# Autodesk Inventor assembly: Full Car Assembly
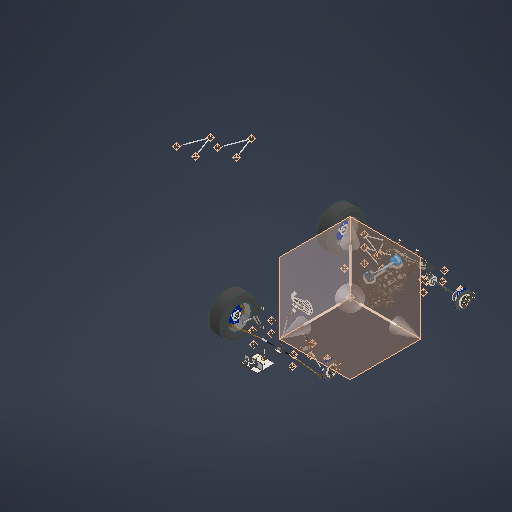
[picture p0: Inventor's stored thumbnail of the model, 512x512]
Saved by Autodesk Inventor 2026.1 (Build 301233000, 233)
## iProperties
Created: 2026-07-07
Part Number: Full Car Assembly
Document SubType Name: Assembly
Designer: share
Mass: 339781 g
Surface Area: 198029 cm^2
Volume: 256393 cm^3
Density: 1.32523 g/cm^3
Author: share
## Documents named in this file (36)
- C:\Users\share\OneDrive\Documents\Personal Projects\GOGO Kart\CAD\GOGO_KART_FSAE\Full Car Assembly.iam
- C:\Users\share\OneDrive\Documents\Personal Projects\GOGO Kart\CAD\GOGO_KART_FSAE\FrameV2\Frame\Frame 1780692296746.iam
- C:\Users\share\OneDrive\Documents\Personal Projects\GOGO Kart\CAD\GOGO_KART_FSAE\Drivetrain\honda-cbr600-f4i-engine-1.snapshot.3\Honda CBR600 F4i\Honda CBR600 F4i\Honda CBR600 F4i.ipt
- C:\Users\share\OneDrive\Documents\Personal Projects\GOGO Kart\CAD\GOGO_KART_FSAE\Shifter\crank.ipt
- C:\Users\share\OneDrive\Documents\Personal Projects\GOGO Kart\CAD\GOGO_KART_FSAE\Shifter\59935K71_Ball Joint Rod End\59935K71_Ball Joint Rod End\59935K71_Ball Joint Rod End.ipt
- C:\Users\share\OneDrive\Documents\Personal Projects\GOGO Kart\CAD\GOGO_KART_FSAE\Shifter\threadedtubeshort.ipt
- C:\Users\share\OneDrive\Documents\Personal Projects\GOGO Kart\CAD\GOGO_KART_FSAE\Shifter\ShifterBracket.ipt
- C:\Users\share\OneDrive\Documents\Personal Projects\GOGO Kart\CAD\GOGO_KART_FSAE\Shifter\BellCrank.ipt
- C:\Users\share\OneDrive\Documents\Personal Projects\GOGO Kart\CAD\GOGO_KART_FSAE\Shifter\Bearing.ipt
- C:\Users\share\OneDrive\Documents\Personal Projects\GOGO Kart\CAD\GOGO_KART_FSAE\Shifter\spacer.ipt
- C:\Users\share\OneDrive\Documents\Personal Projects\GOGO Kart\CAD\GOGO_KART_FSAE\Shifter\6045N121_Low-Carbon Steel Round Tube\6045N121_Low-Carbon Steel Round Tube\6045N121_Low-Carbon Steel Round Tube.ipt
- C:\Users\share\OneDrive\Documents\Inventor\Content Center Files\R2026\en-US\ISO 4032(2)\ISO 4032 - M5 - ISO.ipt
- C:\Users\share\OneDrive\Documents\Personal Projects\GOGO Kart\CAD\GOGO_KART_FSAE\Shifter\stickshift.ipt
- C:\Users\share\OneDrive\Documents\Personal Projects\GOGO Kart\CAD\GOGO_KART_FSAE\Shifter\stickplate.ipt
- C:\Users\share\OneDrive\Documents\Personal Projects\GOGO Kart\CAD\GOGO_KART_FSAE\Suspension\Hardware\ALLSTAR 0.5 in Rod End Bracket (Rough).ipt
- C:\Users\share\OneDrive\Documents\Personal Projects\GOGO Kart\CAD\GOGO_KART_FSAE\Drivetrain\Engine Mounting\Engine_Mount_Reference_Model_V1.ipt
- C:\Users\share\OneDrive\Documents\Personal Projects\GOGO Kart\CAD\GOGO_KART_FSAE\Drivetrain\Left_Engine_Mount_Assembly_V1.iam
- C:\Users\share\OneDrive\Documents\Personal Projects\GOGO Kart\CAD\GOGO_KART_FSAE\Drivetrain\Right_Lower_Engine_Mount_Assembly_V1.iam
- C:\Users\share\OneDrive\Documents\Personal Projects\GOGO Kart\CAD\GOGO_KART_FSAE\Suspension\SpringSetup\largebracket.ipt
- C:\Users\share\OneDrive\Documents\Personal Projects\GOGO Kart\CAD\GOGO_KART_FSAE\Suspension\SpringSetup\ShockAbsorber.ipt
- C:\Users\share\OneDrive\Documents\Personal Projects\GOGO Kart\CAD\GOGO_KART_FSAE\Suspension\SpringSetup\RockerFront.ipt
- C:\Users\share\OneDrive\Documents\Personal Projects\GOGO Kart\CAD\GOGO_KART_FSAE\Suspension\SpringSetup\sus_rods.ipt
- C:\Users\share\OneDrive\Documents\Personal Projects\GOGO Kart\CAD\GOGO_KART_FSAE\Suspension\Suspension Arms\Suspension Rod Ends\5-8 Rod End Assembly.iam
- C:\Users\share\OneDrive\Documents\Personal Projects\GOGO Kart\CAD\GOGO_KART_FSAE\Suspension\SpringSetup\RockerRear.ipt
- C:\Users\share\OneDrive\Documents\Personal Projects\GOGO Kart\CAD\GOGO_KART_FSAE\Suspension\SpringSetup\susrod_rear.ipt
- C:\Users\share\OneDrive\Documents\Personal Projects\GOGO Kart\CAD\GOGO_KART_FSAE\Steering\SteeringAssy.iam
- C:\Users\share\OneDrive\Documents\Personal Projects\GOGO Kart\CAD\GOGO_KART_FSAE\Steering\steeringmountplate.ipt
- C:\Users\share\OneDrive\Documents\Personal Projects\GOGO Kart\CAD\GOGO_KART_FSAE\Steering\steeringbracket.ipt
- C:\Users\share\OneDrive\Documents\Personal Projects\GOGO Kart\CAD\GOGO_KART_FSAE\Steering\rackbracket.ipt
- C:\Users\share\OneDrive\Documents\Personal Projects\GOGO Kart\CAD\GOGO_KART_FSAE\Steering\rackmountplate.ipt
- C:\Users\share\OneDrive\Documents\Personal Projects\GOGO Kart\CAD\GOGO_KART_FSAE\Drivetrain\Diff_Assembly_V1.iam
- C:\Users\share\OneDrive\Documents\Personal Projects\GOGO Kart\CAD\GOGO_KART_FSAE\Drivetrain\CV Axles\Porsche_912_Standard_CV_Axle_Assembly.iam
- C:\Users\share\OneDrive\Documents\Personal Projects\GOGO Kart\CAD\GOGO_KART_FSAE\Suspension\REAL Upright\V2\Upright_Assembly_V2.iam
- C:\Users\share\Downloads\Driver CAD Model.iam
- C:\Users\share\OneDrive\Documents\Personal Projects\GOGO Kart\CAD\GOGO_KART_FSAE\Pedal Box\Pedal_Box_V2_Test\Pedalbox_V2_Assembly.iam
- C:\Users\share\OneDrive\Documents\Personal Projects\GOGO Kart\CAD\GOGO_KART_FSAE\Suspension\Suspension_Arm_V2\Suspenion_Arm_Assembly_V2.iam
## Components (93 placed, 35 different names)
1. Porsche_912_Standard_CV_Axle_Assembly:1 [sub-assembly] — Mate:66, Rigid:6, Mate:71
2. Porsche_912_Standard_CV_Axle_Assembly:2 [sub-assembly] — Mate:67, Mate:68, Mate:70
3. Upright_Assembly_V2:1 [sub-assembly] — Angle:33
4. Upright_Assembly_V2:2 [sub-assembly] — Angle:32
5. Upright_Assembly_V2:3 [sub-assembly] — Angle:35, Mate:70
6. Upright_Assembly_V2:4 [sub-assembly] — Angle:34, Mate:71
7. Driver CAD Model:1 [sub-assembly]
8. Pedalbox_V2_Assembly:1 [sub-assembly] — Tangent:36, Tangent:37, Mate:72
9. Suspenion_Arm_Assembly_V2:1 [sub-assembly] — Mate:73, Mate:74
10. Suspenion_Arm_Assembly_V2:2 [sub-assembly] — Mate:75, Mate:76
11. Suspenion_Arm_Assembly_V2:3 [sub-assembly]
12. Suspenion_Arm_Assembly_V2:4 [sub-assembly]
13. Porsche_912_Standard_CV_Axle_Assembly:3 [sub-assembly]
14. Frame 1780692296746:1 [sub-assembly] — Flush:1, Flush:2, Flush:3, Tangent:1, Tangent:2, Front Left: LF Floor Mate, Front Left: LF Front Mate, Front Left: LF Tangent Mate, Front Left: LR Floor Mate, Front Left: LR Front Mate, Front Left: LR Tangent Mate, Front Left: UF Floor Mate, Front Left: UF Front Mate, Front Left: UF Tangent Mate, Front Left: UR Floor Mate, Front Left: UR Front Mate, Front Left: UR Tangent Mate, Rear Left: LF Floor Mate, Rear Left: LF Front Mate, Rear Left: LF Tangent Mate, Rear Left: LR Floor Mate, Rear Left: LR Front Mate, Rear Left: LR Tangent Mate, Rear Left: UF Floor Mate, Rear Left: UF Front Mate, Rear Left: UF Tangent Mate, Rear Left: UR Floor Mate, Rear Left: UR Front Mate, Rear Left: UR Tangent Mate, Front Right: LF Floor Mate, Front Right: LF Front Mate, Front Right: LF Tangent  Mate, Front Right: LR Floor Mate, Front Right: LR Front Mate, Front Right: LR Tangent  Mate, Front Right: UF Floor Mate, Front Right: UF Front Mate, Front Right: UF Tangent Mate, Front Right: UR Floor Mate, Front Right: UR Front Mate, Front Right: UR Tangent  Mate, Rear Right: LF Floor Mate, Rear Right: LF Front Mate, Rear Right: LF Tangent Mate, Rear Right: LR Floor Mate, Rear Right: LR Front Mate, Rear Right: LR Tangent Mate, Rear Right: UR Floor Mate, Rear Right: UR Front Mate, Rear Ritgh: UR Tangent Mate, Rear Right: UF Floor Mate, Rear Right: UF Front Mate, Rear Rigth: UF Tangent Mate, Engine Reference Horizontal Mate, Engine Reference Vertical Mate, Insert:3, Angle:2, Insert:4, Angle:4, Angle:6, Angle:7, Insert:6, Insert:7, Tangent:19, Mate:39, Tangent:20, Mate:40, Tangent:21, Tangent:22, Tangent:23, Tangent:24, Tangent:25, Tangent:28, Tangent:30, Tangent:31, Mate:54, Tangent:33, Tangent:34, Mate:69, Tangent:35, Tangent:36, Tangent:37
15. stickshift:1 — Rigid:4
16. stickplate:1 — Rigid:4, Tangent:2
17. crank:1 — Insert:2
18. 59935K71_Ball Joint Rod End:1 — Rotational:2, Angle:1, Rotational:6
19. 59935K71_Ball Joint Rod End:3 — Insert:2, Rotational:1, Angle:1
20. threadedtubeshort:1 — Rotational:1, Rotational:2
21. ShifterBracket:1 — Rigid:1, Tangent:1
22. BellCrank:1 — Rotational:3, Rotational:6
23. Bearing:1 — Rotational:3, Rotational:4, Rotational:5
24. spacer:1 — Rigid:1, Rotational:4
25. spacer:2 — Rotational:5
26. 6045N121_Low-Carbon Steel Round Tube:1 — Rigid:2, Rigid:3
27. ISO 4032 M5:1 — Rigid:3
28. ISO 4032 M5:2 — Rigid:2
29. 5-8 Rod End Assembly:7 [sub-assembly] — Rotational:77, Angle:25
30. 5-8 Rod End Assembly:8 [sub-assembly] — Rotational:78, Angle:27
31. ALLSTAR 0.5 in Rod End Bracket (Rough):23 — Rotational:78, Angle:27
32. 5-8 Rod End Assembly:3 [sub-assembly] — Rotational:57, Rotational:59
33. 5-8 Rod End Assembly:4 [sub-assembly] — Rotational:58, Rotational:61, Angle:15, Angle:16
34. ALLSTAR 0.5 in Rod End Bracket (Rough):20 — Angle:12
35. ALLSTAR 0.5 in Rod End Bracket (Rough):21 — Rotational:61, Angle:15
36. 5-8 Rod End Assembly:5 [sub-assembly] — Rotational:69, Angle:20
37. 5-8 Rod End Assembly:6 [sub-assembly] — Angle:19, Rotational:70
38. ALLSTAR 0.5 in Rod End Bracket (Rough):22 — Rotational:69, Angle:20, Angle:21
39. largebracket:8 — Tangent:30, Angle:22, Mate:50, Mate:51, Rotational:71
40. largebracket:9 — Angle:23, Tangent:31, Mate:52, Rotational:72, Rotational:73
41. RockerRear:3 — Rotational:72, Angle:24, Rotational:74, Rotational:77, Angle:25
42. RockerRear:4 — Rotational:73, Angle:24
43. susrod_rear:2
44. largebracket:7 — Mate:49, Angle:17, Tangent:28, Rotational:62
45. ShockAbsorber:3 — Rotational:62, Rotational:65
46. ShockAbsorber:4 — Rotational:71, Rotational:74
47. RockerFront:4 — Rotational:64, Angle:18, Rotational:65, Angle:21, Rotational:70
48. RockerFront:5 — Rotational:63, Angle:18, Angle:19
49. sus_rods:2
50. largebracket:5 — Tangent:24, Angle:9, Mate:46, Mate:47, Rotational:55, Angle:22
51. largebracket:6 — Angle:10, Tangent:25, Mate:48, Rotational:53, Rotational:54, Angle:23
52. RockerRear:1 — Rotational:53, Angle:11, Rotational:59, Angle:16
53. RockerRear:2 — Rotational:54, Angle:11, Rotational:56
54. ShockAbsorber:2 — Rotational:55, Rotational:56
55. susrod_rear:1 — Rotational:57, Rotational:58
56. largebracket:1 — Tangent:21, Mate:41, Mate:42, Rotational:42, Rotational:43
57. largebracket:2 — Tangent:22, Mate:43, Mate:44, Angle:17, Rotational:63, Rotational:64
58. largebracket:4 — Tangent:23, Mate:45, Rotational:41
59. ShockAbsorber:1 — Rotational:41, Rotational:44
60. RockerFront:2 — Rotational:42, Angle:8, Rotational:44, Angle:12
61. RockerFront:3 — Rotational:43, Angle:8
62. sus_rods:1
63. ALLSTAR 0.5 in Rod End Bracket (Rough):1 — Front Left: LF Floor Mate, Front Left: LF Front Mate, Front Left: LF Tangent Mate
64. ALLSTAR 0.5 in Rod End Bracket (Rough):2 — Front Left: LR Floor Mate, Front Left: LR Front Mate, Front Left: LR Tangent Mate
65. ALLSTAR 0.5 in Rod End Bracket (Rough):3 — Front Left: UF Floor Mate, Front Left: UF Front Mate, Front Left: UF Tangent Mate, Mate:42
66. ALLSTAR 0.5 in Rod End Bracket (Rough):4 — Front Left: UR Floor Mate, Front Left: UR Front Mate, Front Left: UR Tangent Mate
67. ALLSTAR 0.5 in Rod End Bracket (Rough):5 — Rear Left: LF Floor Mate, Rear Left: LF Front Mate, Rear Left: LF Tangent Mate
68. ALLSTAR 0.5 in Rod End Bracket (Rough):6 — Rear Left: UF Floor Mate, Rear Left: UF Front Mate, Rear Left: UF Tangent Mate
69. ALLSTAR 0.5 in Rod End Bracket (Rough):7 — Rear Left: UR Floor Mate, Rear Left: UR Front Mate, Rear Left: UR Tangent Mate, Angle:9, Angle:10
70. ALLSTAR 0.5 in Rod End Bracket (Rough):8 — Rear Left: LR Floor Mate, Rear Left: LR Front Mate, Rear Left: LR Tangent Mate
71. ALLSTAR 0.5 in Rod End Bracket (Rough):9 — Front Right: LF Floor Mate, Front Right: LF Front Mate, Front Right: LF Tangent  Mate
72. ALLSTAR 0.5 in Rod End Bracket (Rough):10 — Front Right: LR Floor Mate, Front Right: LR Front Mate, Front Right: LR Tangent  Mate
73. ALLSTAR 0.5 in Rod End Bracket (Rough):11 — Front Right: UR Floor Mate, Front Right: UR Front Mate, Front Right: UR Tangent  Mate
74. ALLSTAR 0.5 in Rod End Bracket (Rough):12 — Front Right: UF Floor Mate, Front Right: UF Front Mate, Front Right: UF Tangent Mate, Mate:44
75. ALLSTAR 0.5 in Rod End Bracket (Rough):13 — Rear Right: LF Floor Mate, Rear Right: LF Front Mate, Rear Right: LF Tangent Mate, Mate:76
76. ALLSTAR 0.5 in Rod End Bracket (Rough):14 — Rear Right: LR Floor Mate, Rear Right: LR Front Mate, Rear Right: LR Tangent Mate, Mate:75
77. ALLSTAR 0.5 in Rod End Bracket (Rough):15 — Rear Right: UR Floor Mate, Rear Right: UR Front Mate, Rear Ritgh: UR Tangent Mate, Mate:73
78. ALLSTAR 0.5 in Rod End Bracket (Rough):16 — Rear Right: UF Floor Mate, Rear Right: UF Front Mate, Rear Rigth: UF Tangent Mate, Mate:74
79. Honda CBR600 F4i:1 — Insert:5, Angle:4
80. Engine_Mount_Reference_Model_V1:1 — Engine Reference Horizontal Mate, Engine Reference Vertical Mate
81. ALLSTAR 0.5 in Rod End Bracket (Rough):18 — Tangent:19, Mate:39
82. ALLSTAR 0.5 in Rod End Bracket (Rough):19 — Tangent:20, Mate:40
83. Left_Engine_Mount_Assembly_V1:1 [sub-assembly] — Insert:3, Angle:2, Angle:3, Insert:5
84. Left_Engine_Mount_Assembly_V1:2 [sub-assembly] — Insert:4, Angle:3
85. Right_Lower_Engine_Mount_Assembly_V1:1 [sub-assembly] — Angle:6, Insert:7
86. Right_Lower_Engine_Mount_Assembly_V1:2 [sub-assembly] — Angle:7, Insert:6
87. Diff_Assembly_V1:1 [sub-assembly] — Angle:31, Mate:66, Rigid:6, Mate:67, Mate:68, Mate:69, Tangent:35
88. SteeringAssy:1 [sub-assembly] — Rotational:83, Angle:28, Mate:63, Angle:29, Angle:30
89. steeringmountplate:1 — Mate:53, Mate:54, Mate:55, Rotational:79, Rotational:80
90. steeringbracket:1 — Rotational:79, Rotational:80, Rotational:83
91. rackmountplate:1 — Tangent:33, Tangent:34, Mate:56, Rotational:84, Mate:62, Angle:28, Rotational:85, Mate:64, Angle:29, Angle:30
92. rackbracket:2 — Rotational:84, Mate:62, Mate:63
93. rackbracket:3 — Rotational:85, Mate:64
## Relationships (183: Mate 57, RevoluteJoint 39, Tangent 33, Angle 31, Flush 12, Insert 6, WeldJoint 5)
- Flush:1: Frame 1780692296746:1
- Flush:2: Frame 1780692296746:1
- Flush:3: Frame 1780692296746:1
- Insert:2: crank:1 ↔ 59935K71_Ball Joint Rod End:3
- Rotational:1 [RevoluteJoint]: 59935K71_Ball Joint Rod End:3 ↔ threadedtubeshort:1
- Rotational:2 [RevoluteJoint]: 59935K71_Ball Joint Rod End:1 ↔ threadedtubeshort:1
- Angle:1 (90 deg): 59935K71_Ball Joint Rod End:1 ↔ 59935K71_Ball Joint Rod End:3
- Rigid:1 [WeldJoint]: ShifterBracket:1 ↔ spacer:1
- Rotational:3 [RevoluteJoint]: BellCrank:1 ↔ Bearing:1
- Rotational:4 [RevoluteJoint]: Bearing:1 ↔ spacer:1
- Rotational:5 [RevoluteJoint]: Bearing:1 ↔ spacer:2
- Rotational:6 [RevoluteJoint]: 59935K71_Ball Joint Rod End:1 ↔ BellCrank:1
- Tangent:1: Frame 1780692296746:1 ↔ ShifterBracket:1
- Rigid:2 [WeldJoint]: 6045N121_Low-Carbon Steel Round Tube:1 ↔ ISO 4032 M5:2
- Rigid:3 [WeldJoint]: 6045N121_Low-Carbon Steel Round Tube:1 ↔ ISO 4032 M5:1
- Rigid:4 [WeldJoint]: stickshift:1 ↔ stickplate:1
- Tangent:2: Frame 1780692296746:1 ↔ stickplate:1
- Front Left: LF Floor Mate [Mate] (200 mm): Frame 1780692296746:1 ↔ ALLSTAR 0.5 in Rod End Bracket (Rough):1
- Front Left: LF Front Mate [Flush] (350 mm): Frame 1780692296746:1 ↔ ALLSTAR 0.5 in Rod End Bracket (Rough):1
- Front Left: LF Tangent Mate [Tangent]: Frame 1780692296746:1 ↔ ALLSTAR 0.5 in Rod End Bracket (Rough):1
- Front Left: LR Floor Mate [Mate] (200 mm): Frame 1780692296746:1 ↔ ALLSTAR 0.5 in Rod End Bracket (Rough):2
- Front Left: LR Front Mate [Flush] (610 mm): Frame 1780692296746:1 ↔ ALLSTAR 0.5 in Rod End Bracket (Rough):2
- Front Left: LR Tangent Mate [Tangent]: Frame 1780692296746:1 ↔ ALLSTAR 0.5 in Rod End Bracket (Rough):2
- Front Left: UF Floor Mate [Mate] (350 mm): Frame 1780692296746:1 ↔ ALLSTAR 0.5 in Rod End Bracket (Rough):3
- Front Left: UF Front Mate [Flush] (360 mm): Frame 1780692296746:1 ↔ ALLSTAR 0.5 in Rod End Bracket (Rough):3
- Front Left: UF Tangent Mate [Tangent]: Frame 1780692296746:1 ↔ ALLSTAR 0.5 in Rod End Bracket (Rough):3
- Front Left: UR Floor Mate [Mate] (350 mm): Frame 1780692296746:1 ↔ ALLSTAR 0.5 in Rod End Bracket (Rough):4
- Front Left: UR Front Mate [Flush] (620 mm): Frame 1780692296746:1 ↔ ALLSTAR 0.5 in Rod End Bracket (Rough):4
- Front Left: UR Tangent Mate [Tangent]: Frame 1780692296746:1 ↔ ALLSTAR 0.5 in Rod End Bracket (Rough):4
- Rear Left: LF Floor Mate [Mate] (200 mm): Frame 1780692296746:1 ↔ ALLSTAR 0.5 in Rod End Bracket (Rough):5
- Rear Left: LF Front Mate [Flush] (2180 mm): Frame 1780692296746:1 ↔ ALLSTAR 0.5 in Rod End Bracket (Rough):5
- Rear Left: LF Tangent Mate [Tangent]: Frame 1780692296746:1 ↔ ALLSTAR 0.5 in Rod End Bracket (Rough):5
- Rear Left: LR Floor Mate [Mate] (200 mm): Frame 1780692296746:1 ↔ ALLSTAR 0.5 in Rod End Bracket (Rough):8
- Rear Left: LR Front Mate [Flush] (2440 mm): Frame 1780692296746:1 ↔ ALLSTAR 0.5 in Rod End Bracket (Rough):8
- Rear Left: LR Tangent Mate [Tangent]: Frame 1780692296746:1 ↔ ALLSTAR 0.5 in Rod End Bracket (Rough):8
- Rear Left: UF Floor Mate [Mate] (350 mm): Frame 1780692296746:1 ↔ ALLSTAR 0.5 in Rod End Bracket (Rough):6
- Rear Left: UF Front Mate [Flush] (2180 mm): Frame 1780692296746:1 ↔ ALLSTAR 0.5 in Rod End Bracket (Rough):6
- Rear Left: UF Tangent Mate [Tangent]: Frame 1780692296746:1 ↔ ALLSTAR 0.5 in Rod End Bracket (Rough):6
- Rear Left: UR Floor Mate [Mate] (350 mm): Frame 1780692296746:1 ↔ ALLSTAR 0.5 in Rod End Bracket (Rough):7
- Rear Left: UR Front Mate [Flush] (2440 mm): Frame 1780692296746:1 ↔ ALLSTAR 0.5 in Rod End Bracket (Rough):7
- Rear Left: UR Tangent Mate [Tangent]: Frame 1780692296746:1 ↔ ALLSTAR 0.5 in Rod End Bracket (Rough):7
- Front Right: LF Floor Mate [Mate] (200 mm): Frame 1780692296746:1 ↔ ALLSTAR 0.5 in Rod End Bracket (Rough):9
- Front Right: LF Front Mate [Mate] (-350 mm): Frame 1780692296746:1 ↔ ALLSTAR 0.5 in Rod End Bracket (Rough):9
- Front Right: LF Tangent  Mate [Tangent]: Frame 1780692296746:1 ↔ ALLSTAR 0.5 in Rod End Bracket (Rough):9
- Front Right: LR Floor Mate [Mate] (200 mm): Frame 1780692296746:1 ↔ ALLSTAR 0.5 in Rod End Bracket (Rough):10
- Front Right: LR Front Mate [Mate] (-610 mm): Frame 1780692296746:1 ↔ ALLSTAR 0.5 in Rod End Bracket (Rough):10
- Front Right: LR Tangent  Mate [Tangent]: Frame 1780692296746:1 ↔ ALLSTAR 0.5 in Rod End Bracket (Rough):10
- Front Right: UF Floor Mate [Mate] (350 mm): Frame 1780692296746:1 ↔ ALLSTAR 0.5 in Rod End Bracket (Rough):12
- Front Right: UF Front Mate [Mate] (-360 mm): Frame 1780692296746:1 ↔ ALLSTAR 0.5 in Rod End Bracket (Rough):12
- Front Right: UF Tangent Mate [Tangent]: Frame 1780692296746:1 ↔ ALLSTAR 0.5 in Rod End Bracket (Rough):12
- Front Right: UR Floor Mate [Mate] (350 mm): Frame 1780692296746:1 ↔ ALLSTAR 0.5 in Rod End Bracket (Rough):11
- Front Right: UR Front Mate [Mate] (-620 mm): Frame 1780692296746:1 ↔ ALLSTAR 0.5 in Rod End Bracket (Rough):11
- Front Right: UR Tangent  Mate [Tangent]: Frame 1780692296746:1 ↔ ALLSTAR 0.5 in Rod End Bracket (Rough):11
- Rear Right: LF Floor Mate [Mate] (200 mm): Frame 1780692296746:1 ↔ ALLSTAR 0.5 in Rod End Bracket (Rough):13
- Rear Right: LF Front Mate [Mate] (-2180 mm): Frame 1780692296746:1 ↔ ALLSTAR 0.5 in Rod End Bracket (Rough):13
- Rear Right: LF Tangent Mate [Tangent]: Frame 1780692296746:1 ↔ ALLSTAR 0.5 in Rod End Bracket (Rough):13
- Rear Right: LR Floor Mate [Mate] (200 mm): Frame 1780692296746:1 ↔ ALLSTAR 0.5 in Rod End Bracket (Rough):14
- Rear Right: LR Front Mate [Mate] (-2440 mm): Frame 1780692296746:1 ↔ ALLSTAR 0.5 in Rod End Bracket (Rough):14
- Rear Right: LR Tangent Mate [Tangent]: Frame 1780692296746:1 ↔ ALLSTAR 0.5 in Rod End Bracket (Rough):14
- Rear Right: UR Floor Mate [Mate] (350 mm): Frame 1780692296746:1 ↔ ALLSTAR 0.5 in Rod End Bracket (Rough):15
- Rear Right: UR Front Mate [Mate] (-2440 mm): Frame 1780692296746:1 ↔ ALLSTAR 0.5 in Rod End Bracket (Rough):15
- Rear Ritgh: UR Tangent Mate [Tangent]: Frame 1780692296746:1 ↔ ALLSTAR 0.5 in Rod End Bracket (Rough):15
- Rear Right: UF Floor Mate [Mate] (350 mm): Frame 1780692296746:1 ↔ ALLSTAR 0.5 in Rod End Bracket (Rough):16
- Rear Right: UF Front Mate [Mate] (-2180 mm): Frame 1780692296746:1 ↔ ALLSTAR 0.5 in Rod End Bracket (Rough):16
- Rear Rigth: UF Tangent Mate [Tangent]: Frame 1780692296746:1 ↔ ALLSTAR 0.5 in Rod End Bracket (Rough):16
- Engine Reference Horizontal Mate [Mate] (30 mm): Frame 1780692296746:1 ↔ Engine_Mount_Reference_Model_V1:1
- Engine Reference Vertical Mate [Flush] (400 mm): Frame 1780692296746:1 ↔ Engine_Mount_Reference_Model_V1:1
- Insert:3: Frame 1780692296746:1 ↔ Left_Engine_Mount_Assembly_V1:1
- Angle:2 (0 deg): Frame 1780692296746:1 ↔ Left_Engine_Mount_Assembly_V1:1
- Insert:4: Frame 1780692296746:1 ↔ Left_Engine_Mount_Assembly_V1:2
- Angle:3 (0 deg): Left_Engine_Mount_Assembly_V1:1 ↔ Left_Engine_Mount_Assembly_V1:2
- Insert:5: Honda CBR600 F4i:1 ↔ Left_Engine_Mount_Assembly_V1:1
- Angle:4 (0 deg): Frame 1780692296746:1 ↔ Honda CBR600 F4i:1
- Angle:6 (0 deg): Frame 1780692296746:1 ↔ Right_Lower_Engine_Mount_Assembly_V1:1
- Angle:7 (0 deg): Frame 1780692296746:1 ↔ Right_Lower_Engine_Mount_Assembly_V1:2
- Insert:6: Frame 1780692296746:1 ↔ Right_Lower_Engine_Mount_Assembly_V1:2
- Insert:7: Frame 1780692296746:1 ↔ Right_Lower_Engine_Mount_Assembly_V1:1
- Tangent:19: Frame 1780692296746:1 ↔ ALLSTAR 0.5 in Rod End Bracket (Rough):18
- Mate:39 (400 mm): Frame 1780692296746:1 ↔ ALLSTAR 0.5 in Rod End Bracket (Rough):18
- Tangent:20: Frame 1780692296746:1 ↔ ALLSTAR 0.5 in Rod End Bracket (Rough):19
- Mate:40 (450 mm): Frame 1780692296746:1 ↔ ALLSTAR 0.5 in Rod End Bracket (Rough):19
- Tangent:21: Frame 1780692296746:1 ↔ largebracket:1
- Mate:41 (350 mm): largebracket:1
- Mate:42 (-105 mm): largebracket:1 ↔ ALLSTAR 0.5 in Rod End Bracket (Rough):3
- Tangent:22: Frame 1780692296746:1 ↔ largebracket:2
- Mate:43 (350 mm): largebracket:2
- Mate:44 (145 mm): largebracket:2 ↔ ALLSTAR 0.5 in Rod End Bracket (Rough):12
- Tangent:23: Frame 1780692296746:1 ↔ largebracket:4
- Mate:45 (590 mm): largebracket:4
- Rotational:41 [RevoluteJoint] (-9 mm): largebracket:4 ↔ ShockAbsorber:1
- Rotational:42 [RevoluteJoint]: largebracket:1 ↔ RockerFront:2
- Rotational:43 [RevoluteJoint]: largebracket:1 ↔ RockerFront:3
- Angle:8 (0 deg): RockerFront:2 ↔ RockerFront:3
- Rotational:44 [RevoluteJoint] (6.5 mm): ShockAbsorber:1 ↔ RockerFront:2
- Tangent:24: Frame 1780692296746:1 ↔ largebracket:5
- Angle:9 (0 deg): largebracket:5 ↔ ALLSTAR 0.5 in Rod End Bracket (Rough):7
- Mate:46 (-846 mm): largebracket:5
- Mate:47 (120 mm): largebracket:5
- Angle:10 (180 deg): largebracket:6 ↔ ALLSTAR 0.5 in Rod End Bracket (Rough):7
- Tangent:25: Frame 1780692296746:1 ↔ largebracket:6
- Mate:48 (280 mm): largebracket:6
- Rotational:53 [RevoluteJoint]: largebracket:6 ↔ RockerRear:1
- Rotational:54 [RevoluteJoint]: largebracket:6 ↔ RockerRear:2
- Angle:11 (0 deg): RockerRear:1 ↔ RockerRear:2
- Rotational:55 [RevoluteJoint] (-8.5 mm): largebracket:5 ↔ ShockAbsorber:2
- Rotational:56 [RevoluteJoint] (6 mm): RockerRear:2 ↔ ShockAbsorber:2
- Rotational:57 [RevoluteJoint] (2 mm): 5-8 Rod End Assembly:3 ↔ susrod_rear:1
- Rotational:58 [RevoluteJoint] (-2 mm): 5-8 Rod End Assembly:4 ↔ susrod_rear:1
- Rotational:59 [RevoluteJoint] (6.5 mm): 5-8 Rod End Assembly:3 ↔ RockerRear:1
- Angle:12 (0 deg): ALLSTAR 0.5 in Rod End Bracket (Rough):20 ↔ RockerFront:2
- Rotational:61 [RevoluteJoint]: 5-8 Rod End Assembly:4 ↔ ALLSTAR 0.5 in Rod End Bracket (Rough):21
- Angle:15 (0 deg): 5-8 Rod End Assembly:4 ↔ ALLSTAR 0.5 in Rod End Bracket (Rough):21
- Angle:16 (0 deg): 5-8 Rod End Assembly:4 ↔ RockerRear:1
- Mate:49 (590 mm): largebracket:7
- Angle:17 (180 deg): largebracket:7 ↔ largebracket:2
- Tangent:28: Frame 1780692296746:1 ↔ largebracket:7
- Rotational:62 [RevoluteJoint] (-9 mm): largebracket:7 ↔ ShockAbsorber:3
- Rotational:63 [RevoluteJoint]: RockerFront:5 ↔ largebracket:2
- Rotational:64 [RevoluteJoint]: RockerFront:4 ↔ largebracket:2
- Angle:18 (0 deg): RockerFront:4 ↔ RockerFront:5
- Rotational:65 [RevoluteJoint] (6.5 mm): ShockAbsorber:3 ↔ RockerFront:4
- [RevoluteJoint] (-2 mm): 5-8 Rod End Assembly:5 ↔ sus_rods:2
- [RevoluteJoint] (2 mm): 5-8 Rod End Assembly:6 ↔ sus_rods:2
- Angle:19 (0 deg): 5-8 Rod End Assembly:6 ↔ RockerFront:5
- Rotational:69 [RevoluteJoint]: 5-8 Rod End Assembly:5 ↔ ALLSTAR 0.5 in Rod End Bracket (Rough):22
- Angle:20 (0 deg): 5-8 Rod End Assembly:5 ↔ ALLSTAR 0.5 in Rod End Bracket (Rough):22
- Angle:21 (0 deg): ALLSTAR 0.5 in Rod End Bracket (Rough):22 ↔ RockerFront:4
- Rotational:70 [RevoluteJoint] (6.5 mm): 5-8 Rod End Assembly:6 ↔ RockerFront:4
- Tangent:30: Frame 1780692296746:1 ↔ largebracket:8
- Angle:22 (0 deg): largebracket:8 ↔ largebracket:5
- Mate:50 (-846 mm): largebracket:8
- Mate:51 (-120 mm): largebracket:8
- Angle:23 (0 deg): largebracket:9 ↔ largebracket:6
- Tangent:31: Frame 1780692296746:1 ↔ largebracket:9
- Mate:52 (-280 mm): largebracket:9
- Rotational:71 [RevoluteJoint] (-8.5 mm): largebracket:8 ↔ ShockAbsorber:4
- Rotational:72 [RevoluteJoint]: largebracket:9 ↔ RockerRear:3
- Rotational:73 [RevoluteJoint]: largebracket:9 ↔ RockerRear:4
- Angle:24 (0 deg): RockerRear:3 ↔ RockerRear:4
- Rotational:74 [RevoluteJoint] (6.5 mm): RockerRear:3 ↔ ShockAbsorber:4
- [RevoluteJoint] (2 mm): 5-8 Rod End Assembly:7 ↔ susrod_rear:2
- [RevoluteJoint] (-2 mm): 5-8 Rod End Assembly:8 ↔ susrod_rear:2
- Rotational:77 [RevoluteJoint] (6 mm): 5-8 Rod End Assembly:7 ↔ RockerRear:3
- Angle:25 (0 deg): 5-8 Rod End Assembly:7 ↔ RockerRear:3
- Rotational:78 [RevoluteJoint]: 5-8 Rod End Assembly:8 ↔ ALLSTAR 0.5 in Rod End Bracket (Rough):23
- Angle:27 (0 deg): 5-8 Rod End Assembly:8 ↔ ALLSTAR 0.5 in Rod End Bracket (Rough):23
- Mate:53 (-60 mm): steeringmountplate:1
- Mate:54: Frame 1780692296746:1 ↔ steeringmountplate:1
- Mate:55 (697 mm): steeringmountplate:1
- Rotational:79 [RevoluteJoint]: steeringmountplate:1 ↔ steeringbracket:1
- Rotational:80 [RevoluteJoint]: steeringmountplate:1 ↔ steeringbracket:1
- Tangent:33: Frame 1780692296746:1 ↔ rackmountplate:1
- Tangent:34: Frame 1780692296746:1 ↔ rackmountplate:1
- Mate:56 (-70 mm): rackmountplate:1
- Rotational:83 [RevoluteJoint]: SteeringAssy:1 ↔ steeringbracket:1
- Rotational:84 [RevoluteJoint]: rackmountplate:1 ↔ rackbracket:2
- Mate:62: rackmountplate:1 ↔ rackbracket:2
- Angle:28 (180 deg): SteeringAssy:1 ↔ rackmountplate:1
- Mate:63: SteeringAssy:1 ↔ rackbracket:2
- Rotational:85 [RevoluteJoint]: rackmountplate:1 ↔ rackbracket:3
- Mate:64: rackmountplate:1 ↔ rackbracket:3
- Angle:29 (173 deg): SteeringAssy:1 ↔ rackmountplate:1
- Angle:30 (187 deg): SteeringAssy:1 ↔ rackmountplate:1
- Angle:31 (0 deg): Diff_Assembly_V1:1
- Mate:66: Porsche_912_Standard_CV_Axle_Assembly:1 ↔ Diff_Assembly_V1:1
- Rigid:6 [WeldJoint]: Porsche_912_Standard_CV_Axle_Assembly:1 ↔ Diff_Assembly_V1:1
- Mate:67: Porsche_912_Standard_CV_Axle_Assembly:2 ↔ Diff_Assembly_V1:1
- Mate:68 (250 mm): Porsche_912_Standard_CV_Axle_Assembly:2 ↔ Diff_Assembly_V1:1
- Mate:69: Frame 1780692296746:1 ↔ Diff_Assembly_V1:1
- Tangent:35: Frame 1780692296746:1 ↔ Diff_Assembly_V1:1
- Angle:32 (180 deg): Upright_Assembly_V2:2
- Angle:33 (0 deg): Upright_Assembly_V2:1
- Angle:34 (0 deg): Upright_Assembly_V2:4
- Angle:35 (180 deg): Upright_Assembly_V2:3
- Mate:70: Porsche_912_Standard_CV_Axle_Assembly:2 ↔ Upright_Assembly_V2:3
- Mate:71: Porsche_912_Standard_CV_Axle_Assembly:1 ↔ Upright_Assembly_V2:4
- Tangent:36: Pedalbox_V2_Assembly:1 ↔ Frame 1780692296746:1
- Tangent:37: Pedalbox_V2_Assembly:1 ↔ Frame 1780692296746:1
- Mate:72: Pedalbox_V2_Assembly:1
- Mate:73: Suspenion_Arm_Assembly_V2:1 ↔ ALLSTAR 0.5 in Rod End Bracket (Rough):15
- Mate:74: Suspenion_Arm_Assembly_V2:1 ↔ ALLSTAR 0.5 in Rod End Bracket (Rough):16
- Mate:75: Suspenion_Arm_Assembly_V2:2 ↔ ALLSTAR 0.5 in Rod End Bracket (Rough):14
- Mate:76: Suspenion_Arm_Assembly_V2:2 ↔ ALLSTAR 0.5 in Rod End Bracket (Rough):13
## Named parameters: d349_d280 = -2 mm, d350_d281 = 144.664159 deg, d351_d282 = 2 mm, d352_d283 = -84.74866 deg, d379_d319 = 2 mm, d380_d320 = 89.261446 deg, d381_d321 = -2 mm, d382_d322 = 89.261446 deg
